# Autodesk Inventor assembly: Assembly4
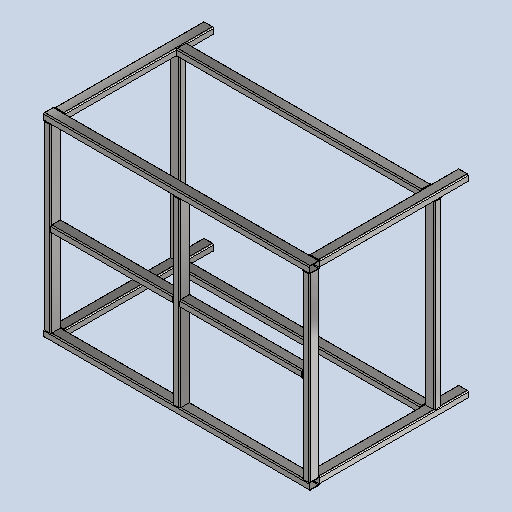
[picture p0: Inventor's stored thumbnail of the model, 512x512]
Saved by Autodesk Inventor 2025 (Build 290162010, 162A)
## iProperties
Created: 2024-09-20
Part Number: Assembly4
Document SubType Name: Assembly
Designer: admin
Author: admin
## Documents named in this file (4)
- C:\Users\admin\YandexDisk-badmisterfox\домашниий пк\Inventor\BSH_Beshkino_bio_tank\Assembly4.iam
- C:\Users\admin\YandexDisk-badmisterfox\домашниий пк\Inventor\BSH_Beshkino_bio_tank\Тумба 2.iam
- C:\Users\admin\YandexDisk-badmisterfox\домашниий пк\Inventor\BSH_Beshkino_bio_tank\Ноги тумба 2.iam
- C:\Users\admin\YandexDisk-badmisterfox\домашниий пк\Inventor\BSH_Beshkino_bio_tank\ISO 4019 - 60x40x3 - 1380.ipt
## Components (5 placed, 3 different names)
1. Тумба 2:1 [sub-assembly]
2. Ноги тумба 2:1 [sub-assembly]
3. Ноги тумба 2:2 [sub-assembly]
4. ISO 4019 - 60x40x3 - 1380:1
5. ISO 4019 - 60x40x3 - 1380:2
## Relationships (10: Flush 6, Mate 3, WeldJoint 1)
- [Mate]: Ноги тумба 2:2 ↔ ISO 4019 - 60x40x3 - 1380:1
- [Flush]: Ноги тумба 2:2 ↔ ISO 4019 - 60x40x3 - 1380:1
- [Flush] (150 mm): Ноги тумба 2:2 ↔ ISO 4019 - 60x40x3 - 1380:1
- [Mate]: Ноги тумба 2:2 ↔ ISO 4019 - 60x40x3 - 1380:2
- [Flush]: Ноги тумба 2:2 ↔ ISO 4019 - 60x40x3 - 1380:2
- [Flush] (150 mm): Ноги тумба 2:2 ↔ ISO 4019 - 60x40x3 - 1380:2
- [Flush]: Ноги тумба 2:1 ↔ Ноги тумба 2:2
- [Flush]: Ноги тумба 2:1 ↔ Ноги тумба 2:2
- [Mate] (1380 mm): Ноги тумба 2:1 ↔ Ноги тумба 2:2
- [WeldJoint]: Тумба 2:1 ↔ Ноги тумба 2:1
